# Autodesk Inventor assembly: 組合檔
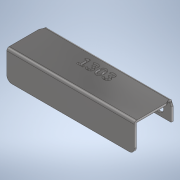
[picture p0: Inventor's stored thumbnail of the model, 180x180]
Saved by Autodesk Inventor 2020 (Build 240168000, 168)
## iProperties
Created: 2015-11-28
Part Number: 組合檔
Document SubType Name: Assembly
Designer: 設計製圖
Author: 設計製圖
## Documents named in this file (3)
- D:\資料庫\設計-3D Project\【May club 】\得利卡-車頂燈架\模型、圖面\22.01.05_設變 (未生產 )\ㄇ槽(#01.05)- 焊接組合.iam
- D:\資料庫\設計-3D Project\【May club 】\得利卡-車頂燈架\模型、圖面\22.01.05_設變 (未生產 )\ㄇ槽-焊接件-1(#01.05).ipt
- D:\資料庫\設計-3D Project\【May club 】\得利卡-車頂燈架\模型、圖面\22.01.05_設變 (未生產 )\ㄇ槽-焊接件-2(#01.05).ipt
## Components (2 placed, 2 different names)
1. ㄇ槽-焊接件-1(#01.05):1 — 貼合:1, 齊平:1, 齊平:2
2. ㄇ槽-焊接件-2(#01.05):1 — 貼合:1, 齊平:1, 齊平:2
## Relationships (3: Flush 2, Mate 1)
- 貼合:1 [Mate]: ㄇ槽-焊接件-1(#01.05):1 ↔ ㄇ槽-焊接件-2(#01.05):1
- 齊平:1 [Flush]: ㄇ槽-焊接件-1(#01.05):1 ↔ ㄇ槽-焊接件-2(#01.05):1
- 齊平:2 [Flush]: ㄇ槽-焊接件-1(#01.05):1 ↔ ㄇ槽-焊接件-2(#01.05):1
